# Autodesk Inventor assembly: Swing_Arm_04
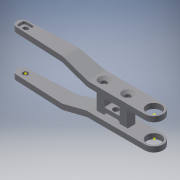
[picture p0: Inventor's stored thumbnail of the model, 180x180]
Saved by Autodesk Inventor 2016 (Build 200138000, 138)
## iProperties
Created: 2016-02-09
Part Number: Swing_Arm_04
Document SubType Name: Assembly
Designer: nils
Author: nils
## Documents named in this file (9)
- D:\bikair\Bikair_CAD-1\Source\Rear_Train\Swing_Arm_04.iam
- D:\bikair\Bikair_CAD-1\Source\Rear_Train\Profile_Straight_04.ipt
- D:\bikair\Bikair_CAD-1\Source\Rear_Train\Profile_Middle_04.ipt
- D:\bikair\Bikair_CAD-1\Source\Rear_Train\Swing_Arm_04\AIP\FEA\boqvscphc.fins
- D:\bikair\Bikair_CAD-1\Source\Rear_Train\Swing_Arm_04\AIP\FEA\boqvscpwg.fsat
- D:\bikair\Bikair_CAD-1\Source\Rear_Train\Swing_Arm_04\AIP\FEA\boqvscq68.ftes
- D:\bikair\Bikair_CAD-1\Source\Rear_Train\Swing_Arm_04\AIP\FEA\boqvscq74.fwiz
- D:\bikair\Bikair_CAD-1\Source\Rear_Train\Swing_Arm_04\AIP\FEA\boqvscrcw.fmsh
- D:\bikair\Bikair_CAD-1\Source\Rear_Train\Swing_Arm_04\AIP\FEA\boqvscrds.fres
## Components (3 placed, 2 different names)
1. Profile_Straight_04:1 — Mate:4, Mate:5, Mate:6
2. Profile_Straight_04:2 — Mate:1, Mate:2, Mate:3
3. Profile_Middle_04:1 — Mate:1, Mate:2, Mate:3, Mate:4, Mate:5, Mate:6
## Relationships (6: Mate 6)
- Mate:1: Profile_Straight_04:2 ↔ Profile_Middle_04:1
- Mate:2: Profile_Straight_04:2 ↔ Profile_Middle_04:1
- Mate:3: Profile_Straight_04:2 ↔ Profile_Middle_04:1
- Mate:4: Profile_Straight_04:1 ↔ Profile_Middle_04:1
- Mate:5: Profile_Straight_04:1 ↔ Profile_Middle_04:1
- Mate:6: Profile_Straight_04:1 ↔ Profile_Middle_04:1
## Named parameters: sa_0 = 2.22e-11, sa_1 = 400000, sa_2 = 7.7e-11, sa_3 = 1.11e-11, sa_4 = -400000, sa_5 = -6.66e-11
note: some values were not read from the file. Shown as the stored number, unit unknown: "sa_0", "sa_1", "sa_2", "sa_3", "sa_4", "sa_5".
